# Autodesk Inventor assembly: FrontFeed
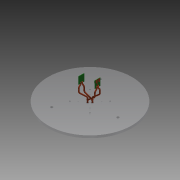
[picture p0: Inventor's stored thumbnail of the model, 180x180]
Saved by Autodesk Inventor 2014 (Build 180170000, 170)
## iProperties
Created: 2015-05-01
Part Number: FrontFeed
Document SubType Name: Assembly
Designer: Owner
Author: Owner
## Documents named in this file (5)
- C:\Users\Owner\Documents\APC\FrontEnd\IAM\Dish\FrontFeed.iam
- C:\Users\Owner\Documents\APC\FrontEnd\IAM\Dish\Base_Can.ipt
- C:\Users\Owner\Documents\APC\FrontEnd\IAM\Dish\FeedSplitter.ipt
- C:\Users\Owner\Documents\APC\FrontEnd\IAM\Dish\Balun.ipt
- C:\Users\Owner\Documents\APC\FrontEnd\IAM\Dish\FeedSplitter2.ipt
## Components (11 placed, 4 different names)
1. Base_Can:1
2. FeedSplitter:1
3. FeedSplitter:2
4. FeedSplitter:3
5. FeedSplitter:4
6. Balun:1
7. FeedSplitter2:1
8. FeedSplitter2:2
9. FeedSplitter2:3
10. FeedSplitter2:4
11. Balun:2
## Relationships (16: Mate 16)
- [Mate]: Base_Can:1 ↔ FeedSplitter:1
- [Mate]: Base_Can:1 ↔ FeedSplitter:2
- [Mate]: Base_Can:1 ↔ FeedSplitter:4
- [Mate]: Base_Can:1 ↔ FeedSplitter:3
- [Mate]: Base_Can:1 ↔ FeedSplitter:3
- [Mate]: Base_Can:1 ↔ FeedSplitter:1
- [Mate]: Base_Can:1 ↔ FeedSplitter:2
- [Mate]: Base_Can:1 ↔ FeedSplitter:4
- [Mate]: FeedSplitter:3 ↔ FeedSplitter2:1
- [Mate]: FeedSplitter:2 ↔ FeedSplitter2:2
- [Mate]: FeedSplitter:2 ↔ FeedSplitter2:2
- [Mate]: FeedSplitter:3 ↔ FeedSplitter2:1
- [Mate]: FeedSplitter:4 ↔ FeedSplitter2:3
- [Mate]: FeedSplitter:4 ↔ FeedSplitter2:3
- [Mate]: FeedSplitter:1 ↔ FeedSplitter2:4
- [Mate]: FeedSplitter:1 ↔ FeedSplitter2:4
